# Autodesk Inventor assembly: main_rename
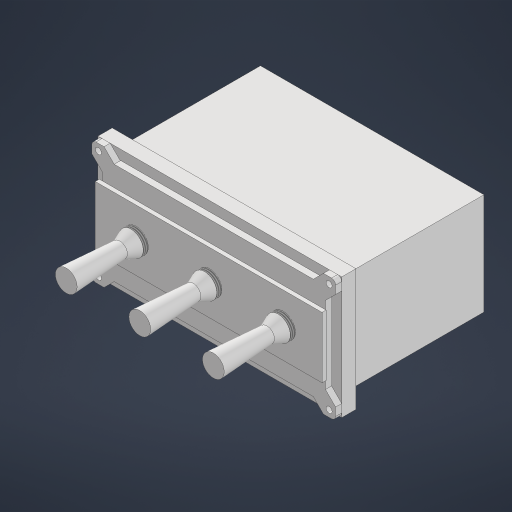
[picture p0: Inventor's stored thumbnail of the model, 512x512]
Saved by Autodesk Inventor 2024 (Build 280153000, 153)
## iProperties
Created: 2026-04-07
Part Number: main_rename
Document SubType Name: Assembly
Designer: schar
Author: schar
## Documents named in this file (5)
- C:\Users\schar\Desktop\MHIPS\models\tiles\2x1\lvl202x01_t\lvl202x01.iam
- C:\Users\schar\Desktop\MHIPS\models\racks\rack_C2x1.ipt
- C:\Users\schar\Desktop\MHIPS\models\tiles\2x1\lvl202x01_t\lvl202x01_toggle_body.ipt
- C:\Users\schar\Desktop\MHIPS\models\switches\NKK_S1AL.ipt
- C:\Users\schar\Desktop\MHIPS\models\switches\lvl2_2x2_guard.ipt
## Components (6 placed, 4 different names)
1. rack_C2x1:1 — Flush:1
2. lvl202x01_toggle_body:1 — Flush:1, Mate:1, Mate:2, Angle:1, Mate:3, Mate:4, Mate:5, Mate:6, Angle:2, Angle:3, Flush:2
3. NKK_S1AL:1 — Mate:1, Mate:2, Angle:1
4. NKK_S1AL:2 — Mate:4, Mate:6, Angle:3
5. NKK_S1AL:3 — Mate:3, Mate:5, Angle:2
6. lvl2_2x2_guard:1 — Flush:2
## Relationships (11: Mate 6, Angle 3, Flush 2)
- Flush:1: rack_C2x1:1 ↔ lvl202x01_toggle_body:1
- Mate:1: lvl202x01_toggle_body:1 ↔ NKK_S1AL:1
- Mate:2: lvl202x01_toggle_body:1 ↔ NKK_S1AL:1
- Angle:1 (0 deg): lvl202x01_toggle_body:1 ↔ NKK_S1AL:1
- Mate:3: lvl202x01_toggle_body:1 ↔ NKK_S1AL:3
- Mate:4: lvl202x01_toggle_body:1 ↔ NKK_S1AL:2
- Mate:5: lvl202x01_toggle_body:1 ↔ NKK_S1AL:3
- Mate:6: lvl202x01_toggle_body:1 ↔ NKK_S1AL:2
- Angle:2 (0 deg): lvl202x01_toggle_body:1 ↔ NKK_S1AL:3
- Angle:3 (0 deg): lvl202x01_toggle_body:1 ↔ NKK_S1AL:2
- Flush:2: lvl202x01_toggle_body:1 ↔ lvl2_2x2_guard:1
